# Autodesk Inventor assembly: PowerDistroPCB_RevC
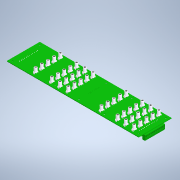
[picture p0: Inventor's stored thumbnail of the model, 180x180]
Saved by Autodesk Inventor 2020.2 (Build 242310000, 310)
## iProperties
Created: 2019-11-25
Part Number: PowerDistroPCB_RevC
Document SubType Name: Assembly
Designer: Rich
Author: Rich
## Documents named in this file (6)
- C:\Users\Rich\development\UWaterloo\power-distro.git\SolidModels\PowerDistroPCB_RevC.iam
- C:\Users\Rich\development\UWaterloo\power-distro.git\SolidModels\power_distro_pcb_RevC.ipt
- C:\Users\Rich\development\UWaterloo\power-distro.git\SolidModels\rcj-021.iam
- C:\Users\Rich\development\UWaterloo\power-distro.git\SolidModels\OST_EDSTLZ950-12.ipt
- C:\Users\Rich\development\UWaterloo\power-distro.git\SolidModels\OST_OSTJ125153.ipt
- C:\Users\Rich\development\UWaterloo\power-distro.git\SolidModels\AAVID_7106.ipt
## Components (46 placed, 5 different names)
1. power_distro_pcb_RevC:1 — Mate:1, Flush:1, Mate:2, Mate:3, Angle:1, Tangent:1, Tangent:2, Mate:4, Mate:5, Mate:6, Tangent:3, Tangent:4, Tangent:5, Tangent:6, Tangent:7, Tangent:8, Angle:2, Angle:3, Angle:4, Mate:7, Angle:5, Mate:8, Angle:6, Flush:2, Flush:3, Flush:4, Flush:5, Flush:6, Flush:7, Mate:13, Angle:7
2. OST_EDSTLZ950-12:1 — Mate:7, Angle:5, Flush:4, Flush:5, Mate:11, Mate:12
3. OST_EDSTLZ950-12:2 — Mate:8, Angle:6, Flush:2, Flush:3, Mate:9, Mate:10
4. OST_OSTJ125153:1 — Mate:9, Mate:10, Flush:6
5. OST_OSTJ125153:2 — Mate:11, Mate:12, Flush:7
6. AAVID_7106:1 — Mate:13, Angle:7
7. rcj-021:1 [sub-assembly] — Mate:3, Angle:1, Tangent:1, Tangent:2
8. rcj-021:2 [sub-assembly] — Mate:5, Tangent:4, Tangent:5, Angle:3
9. rcj-021:3 [sub-assembly] — Mate:4, Tangent:3, Tangent:8, Angle:2
10. rcj-021:4 [sub-assembly] — Mate:6, Tangent:6, Tangent:7, Angle:4
11. rcj-021:5 [sub-assembly]
12. rcj-021:6 [sub-assembly]
13. rcj-021:7 [sub-assembly]
14. rcj-021:8 [sub-assembly]
15. rcj-021:9 [sub-assembly]
16. rcj-021:10 [sub-assembly]
17. rcj-021:11 [sub-assembly]
18. rcj-021:12 [sub-assembly]
19. rcj-021:13 [sub-assembly]
20. rcj-021:14 [sub-assembly]
21. rcj-021:15 [sub-assembly]
22. rcj-021:16 [sub-assembly]
23. rcj-021:17 [sub-assembly]
24. rcj-021:18 [sub-assembly]
25. rcj-021:19 [sub-assembly]
26. rcj-021:20 [sub-assembly]
27. rcj-021:21 [sub-assembly]
28. rcj-021:22 [sub-assembly]
29. rcj-021:23 [sub-assembly]
30. rcj-021:24 [sub-assembly]
31. rcj-021:25 [sub-assembly]
32. rcj-021:26 [sub-assembly]
33. rcj-021:27 [sub-assembly]
34. rcj-021:28 [sub-assembly]
35. rcj-021:29 [sub-assembly]
36. rcj-021:30 [sub-assembly]
37. rcj-021:31 [sub-assembly]
38. rcj-021:32 [sub-assembly]
39. rcj-021:33 [sub-assembly]
40. rcj-021:34 [sub-assembly]
41. rcj-021:35 [sub-assembly]
42. rcj-021:36 [sub-assembly]
43. rcj-021:37 [sub-assembly]
44. rcj-021:38 [sub-assembly]
45. rcj-021:39 [sub-assembly]
46. rcj-021:40 [sub-assembly]
## Component patterns: (10 elements, first: rcj-021:1 + rcj-021:2 + rcj-021:3 + rcj-021:4)
## Relationships (35: Mate 13, Tangent 8, Flush 7, Angle 7)
- Mate:1: power_distro_pcb_RevC:1
- Flush:1: power_distro_pcb_RevC:1
- Mate:2: power_distro_pcb_RevC:1
- Mate:3: power_distro_pcb_RevC:1 ↔ rcj-021:1
- Angle:1 (180 deg): power_distro_pcb_RevC:1 ↔ rcj-021:1
- Tangent:1: power_distro_pcb_RevC:1 ↔ rcj-021:1
- Tangent:2: power_distro_pcb_RevC:1 ↔ rcj-021:1
- Mate:4: power_distro_pcb_RevC:1 ↔ rcj-021:3
- Mate:5: power_distro_pcb_RevC:1 ↔ rcj-021:2
- Mate:6: power_distro_pcb_RevC:1 ↔ rcj-021:4
- Tangent:3: power_distro_pcb_RevC:1 ↔ rcj-021:3
- Tangent:4: power_distro_pcb_RevC:1 ↔ rcj-021:2
- Tangent:5: power_distro_pcb_RevC:1 ↔ rcj-021:2
- Tangent:6: power_distro_pcb_RevC:1 ↔ rcj-021:4
- Tangent:7: power_distro_pcb_RevC:1 ↔ rcj-021:4
- Tangent:8: power_distro_pcb_RevC:1 ↔ rcj-021:3
- Angle:2 (0 deg): power_distro_pcb_RevC:1 ↔ rcj-021:3
- Angle:3 (0 deg): power_distro_pcb_RevC:1 ↔ rcj-021:2
- Angle:4 (0 deg): power_distro_pcb_RevC:1 ↔ rcj-021:4
- Mate:7: power_distro_pcb_RevC:1 ↔ OST_EDSTLZ950-12:1
- Angle:5 (180 deg): power_distro_pcb_RevC:1 ↔ OST_EDSTLZ950-12:1
- Mate:8: power_distro_pcb_RevC:1 ↔ OST_EDSTLZ950-12:2
- Angle:6 (180 deg): power_distro_pcb_RevC:1 ↔ OST_EDSTLZ950-12:2
- Flush:2 (5.207 mm): power_distro_pcb_RevC:1 ↔ OST_EDSTLZ950-12:2
- Flush:3 (23.6474 mm): power_distro_pcb_RevC:1 ↔ OST_EDSTLZ950-12:2
- Flush:4 (23.7744 mm): power_distro_pcb_RevC:1 ↔ OST_EDSTLZ950-12:1
- Flush:5 (10.9982 mm): power_distro_pcb_RevC:1 ↔ OST_EDSTLZ950-12:1
- Mate:9: OST_EDSTLZ950-12:2 ↔ OST_OSTJ125153:1
- Mate:10: OST_EDSTLZ950-12:2 ↔ OST_OSTJ125153:1
- Flush:6 (1.651 mm): power_distro_pcb_RevC:1 ↔ OST_OSTJ125153:1
- Mate:11: OST_EDSTLZ950-12:1 ↔ OST_OSTJ125153:2
- Mate:12: OST_EDSTLZ950-12:1 ↔ OST_OSTJ125153:2
- Flush:7 (1.651 mm): power_distro_pcb_RevC:1 ↔ OST_OSTJ125153:2
- Mate:13: power_distro_pcb_RevC:1 ↔ AAVID_7106:1
- Angle:7 (0 deg): power_distro_pcb_RevC:1 ↔ AAVID_7106:1
